# Autodesk Inventor assembly: 2020Robot
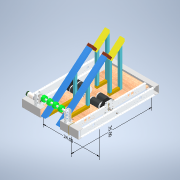
[picture p0: Inventor's stored thumbnail of the model, 180x180]
Saved by Autodesk Inventor 2020.2 (Build 242310000, 310)
## iProperties
Created: 2020-01-26
Part Number: 2020Robot
Document SubType Name: Assembly
Designer: robst
Author: robst
## Documents named in this file (14)
- C:\git\CAD-Development\robSteele\2020CompetitionRobot\2020Robot.iam
- C:\git\CAD-Development\robSteele\2020CompetitionRobot\woodBase.ipt
- C:\git\CAD-Development\robSteele\2020CompetitionRobot\ballRampWithStepForBallLeftSide.iam
- C:\git\CAD-Development\robSteele\2020CompetitionRobot\ballRampWithStepForBallRightSide.iam
- C:\git\CAD-Development\robSteele\2020CompetitionRobot\am-3312a_Gear Intake Kit Gear Config.iam
- C:\git\CAD-Development\robSteele\2020CompetitionRobot\am-3922 AM14U4 Inside Plate.ipt
- C:\git\CAD-Development\robSteele\2020CompetitionRobot\am-3921 AM14U4 Outside Plate.ipt
- C:\git\CAD-Development\robSteele\2020CompetitionRobot\am-3922 AM14U4 Inside Plate_MIR.ipt
- C:\git\CAD-Development\robSteele\2020CompetitionRobot\am-3921 AM14U4 Outside Plate_MIR.ipt
- C:\git\CAD-Development\robSteele\2020CompetitionRobot\2020 End Plate.ipt
- C:\git\CAD-Development\robSteele\2020CompetitionRobot\2020 Front Plate.ipt
- C:\git\CAD-Development\robSteele\2020CompetitionRobot\2020 Front Plate_MIR.ipt
- C:\git\CAD-Development\robSteele\2020CompetitionRobot\ToughBoxMiniWith2CimMotors.iam
- C:\git\CAD-Development\robSteele\2020CompetitionRobot\ToughBoxMiniWith2CimMotors_MIR.iam
## Components (13 placed, 13 different names)
1. woodBase:1 — Flush:1, Flush:2, Flush:3, Mate:1, Mate:2, Mate:4, Mate:5, Mate:7, Flush:5, Mate:8, Mate:9, Mate:13, Mate:14, Mate:15, Mate:16
2. ballRampWithStepForBallLeftSide:1 [sub-assembly] — Mate:1, Mate:2, Mate:3
3. ballRampWithStepForBallRightSide:1 [sub-assembly] — Mate:4, Mate:5, Flush:4
4. am-3312a_Gear Intake Kit Gear Config:1 [sub-assembly] — Mate:6, Mate:7, Flush:5
5. am-3922 AM14U4 Inside Plate:1 — Mate:8, Flush:10, Mate:9, Flush:11, Flush:12, Mate:10, Insert:1, Insert:2
6. am-3921 AM14U4 Outside Plate:1 — Flush:11, Flush:12, Mate:10, Flush:16
7. am-3922 AM14U4 Inside Plate_MIR:1 — Mate:11, Mate:12, Flush:13, Flush:14
8. am-3921 AM14U4 Outside Plate_MIR:1 — Mate:12, Flush:13, Flush:14
9. 2020 End Plate:1 — Flush:15, Mate:13, Mate:14
10. 2020 Front Plate:1 — Mate:15, Mate:16, Flush:16
11. 2020 Front Plate_MIR:1
12. ToughBoxMiniWith2CimMotors:1 [sub-assembly] — Insert:1, Insert:2
13. ToughBoxMiniWith2CimMotors_MIR:1 [sub-assembly]
## Relationships (30: Mate 16, Flush 12, Insert 2)
- Flush:1: woodBase:1
- Flush:2: woodBase:1
- Flush:3: woodBase:1
- Mate:1: woodBase:1 ↔ ballRampWithStepForBallLeftSide:1
- Mate:2: woodBase:1 ↔ ballRampWithStepForBallLeftSide:1
- Mate:3 (57.15 mm): ballRampWithStepForBallLeftSide:1
- Mate:4: woodBase:1 ↔ ballRampWithStepForBallRightSide:1
- Mate:5: woodBase:1 ↔ ballRampWithStepForBallRightSide:1
- Flush:4 (-57.15 mm): ballRampWithStepForBallRightSide:1
- Mate:6: am-3312a_Gear Intake Kit Gear Config:1
- Mate:7 (50.8 mm): woodBase:1 ↔ am-3312a_Gear Intake Kit Gear Config:1
- Flush:5: woodBase:1 ↔ am-3312a_Gear Intake Kit Gear Config:1
- Mate:8: woodBase:1 ↔ am-3922 AM14U4 Inside Plate:1
- Flush:10: am-3922 AM14U4 Inside Plate:1
- Mate:9: woodBase:1 ↔ am-3922 AM14U4 Inside Plate:1
- Flush:11: am-3922 AM14U4 Inside Plate:1 ↔ am-3921 AM14U4 Outside Plate:1
- Flush:12: am-3922 AM14U4 Inside Plate:1 ↔ am-3921 AM14U4 Outside Plate:1
- Mate:10 (85.725 mm): am-3922 AM14U4 Inside Plate:1 ↔ am-3921 AM14U4 Outside Plate:1
- Mate:11: am-3922 AM14U4 Inside Plate_MIR:1
- Mate:12 (85.725 mm): am-3922 AM14U4 Inside Plate_MIR:1 ↔ am-3921 AM14U4 Outside Plate_MIR:1
- Flush:13: am-3922 AM14U4 Inside Plate_MIR:1 ↔ am-3921 AM14U4 Outside Plate_MIR:1
- Flush:14: am-3922 AM14U4 Inside Plate_MIR:1 ↔ am-3921 AM14U4 Outside Plate_MIR:1
- Flush:15: 2020 End Plate:1
- Mate:13: woodBase:1 ↔ 2020 End Plate:1
- Mate:14: woodBase:1 ↔ 2020 End Plate:1
- Mate:15: woodBase:1 ↔ 2020 Front Plate:1
- Mate:16: woodBase:1 ↔ 2020 Front Plate:1
- Flush:16: am-3921 AM14U4 Outside Plate:1 ↔ 2020 Front Plate:1
- Insert:1: am-3922 AM14U4 Inside Plate:1 ↔ ToughBoxMiniWith2CimMotors:1
- Insert:2: am-3922 AM14U4 Inside Plate:1 ↔ ToughBoxMiniWith2CimMotors:1
